# Autodesk Inventor assembly: Motor assembly
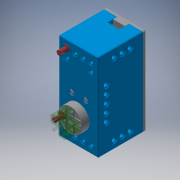
[picture p0: Inventor's stored thumbnail of the model, 180x180]
Saved by Autodesk Inventor 2019 (Build 230136000, 136)
## iProperties
Created: 2018-11-22
Part Number: Motor assembly
Document SubType Name: Assembly
Designer: Varga Daniel
Author: Varga Daniel
## Documents named in this file (11)
- C:\!_Dani\!_cloud\OneDrive\!_munka\Revolution\RevvyDemoKit\Structural parts\Demo parts\Motor\Motor assembly.iam
- C:\!_Dani\!_cloud\OneDrive\!_munka\Revolution\RevvyDemoKit\Structural parts\Demo parts\Motor\FIT0450 motor\FIT0450.iam
- C:\!_Dani\!_cloud\OneDrive\!_munka\Revolution\RevvyDemoKit\Structural parts\Connetor Pins\cp1x1.ipt
- C:\!_Dani\!_cloud\OneDrive\!_munka\Revolution\RevvyDemoKit\Structural parts\Axle Connectors\Axle connector 3x3 cross.ipt
- C:\!_Dani\!_cloud\OneDrive\!_munka\Revolution\RevvyDemoKit\Structural parts\Demo parts\Motor\Motor rotor.ipt
- C:\!_Dani\!_cloud\OneDrive\!_munka\Revolution\RevvyDemoKit\Structural parts\Axles\Axle 2.ipt
- C:\!_Dani\!_cloud\OneDrive\!_dokumentumok\Inventor\Content Center Files\R2019\en-US\ISO 1207(2)\ISO 1207 - M3 x 6.ipt
- C:\!_Dani\!_cloud\OneDrive\!_munka\Revolution\RevvyDemoKit\Structural parts\Demo parts\Motor\Motor cover lower.ipt
- C:\!_Dani\!_cloud\OneDrive\!_dokumentumok\Inventor\Content Center Files\R2019\en-US\ISO 4032(2)\ISO 4032 - M2,5 - ISO.ipt
- C:\!_Dani\!_cloud\OneDrive\!_dokumentumok\Inventor\Content Center Files\R2019\en-US\DIN 7985 (H)\DIN 7985 (H) - M2,5x30-H.ipt
- C:\!_Dani\!_cloud\OneDrive\!_munka\Revolution\RevvyDemoKit\Structural parts\Demo parts\Motor\Motor cover upper.ipt
## Components (15 placed, 10 different names)
1. FIT0450:1 [sub-assembly] — Mate:7, Angle:1, Mate:8, Mate:15, Mate:16, Mate:17, Mate:18, Mate:19, Angle:2
2. cp1x1:1 — Mate:2, Mate:3, Mate:4, Mate:5
3. Axle connector 3x3 cross:1 — Mate:2, Mate:3, Mate:6, Mate:10, Mate:11
4. Motor rotor:1 — Mate:4, Mate:5, Mate:6, Mate:7, Angle:1, Mate:8, Mate:12, Mate:13, Mate:14, Mate:15
5. Axle 2:1 — Mate:10, Mate:11, Mate:14
6. ISO 1207 M3 x 6:1 — Mate:12, Mate:13
7. ISO 4032 M2,5:1 — Mate:16, Mate:17, Flush:2, Flush:3, Angle:2, Angle:3, Angle:4, Flush:4, Mate:20
8. ISO 4032 M2,5:2 — Flush:2, Mate:18, Angle:3, Mate:21, Flush:5
9. ISO 4032 M2,5:3 — Flush:3, Mate:19, Angle:4, Mate:22, Flush:6, Flush:7
10. DIN 7985 (H) M2,5x30-H:1 — Flush:4, Mate:20
11. DIN 7985 (H) M2,5x30-H:2 — Mate:21, Flush:5, Mate:24
12. DIN 7985 (H) M2,5x30-H:3 — Mate:22, Flush:6, Mate:23
13. cp1x1:2 — Mate:26, Mate:27, Mate:28
14. Motor cover lower:1 — Flush:7, Mate:23, Mate:24, Mate:25, Mate:26, Mate:27, Mate:28
15. Motor cover upper:1 — Mate:25
## Relationships (36: Mate 26, Flush 6, Angle 4)
- Mate:2: cp1x1:1 ↔ Axle connector 3x3 cross:1
- Mate:3: cp1x1:1 ↔ Axle connector 3x3 cross:1
- Mate:4: cp1x1:1 ↔ Motor rotor:1
- Mate:5: cp1x1:1 ↔ Motor rotor:1
- Mate:6: Axle connector 3x3 cross:1 ↔ Motor rotor:1
- Mate:7: FIT0450:1 ↔ Motor rotor:1
- Angle:1 (0 deg): FIT0450:1 ↔ Motor rotor:1
- Mate:8: FIT0450:1 ↔ Motor rotor:1
- Mate:10: Axle connector 3x3 cross:1 ↔ Axle 2:1
- Mate:11: Axle connector 3x3 cross:1 ↔ Axle 2:1
- Mate:12: Motor rotor:1 ↔ ISO 1207 M3 x 6:1
- Mate:13: Motor rotor:1 ↔ ISO 1207 M3 x 6:1
- Mate:14: Motor rotor:1 ↔ Axle 2:1
- Mate:15: FIT0450:1 ↔ Motor rotor:1
- Mate:16: FIT0450:1 ↔ ISO 4032 M2,5:1
- Mate:17 (3.5 mm): FIT0450:1 ↔ ISO 4032 M2,5:1
- Flush:2: ISO 4032 M2,5:1 ↔ ISO 4032 M2,5:2
- Mate:18: FIT0450:1 ↔ ISO 4032 M2,5:2
- Flush:3: ISO 4032 M2,5:1 ↔ ISO 4032 M2,5:3
- Mate:19: FIT0450:1 ↔ ISO 4032 M2,5:3
- Angle:2 (0 deg): FIT0450:1 ↔ ISO 4032 M2,5:1
- Angle:3 (0 deg): ISO 4032 M2,5:1 ↔ ISO 4032 M2,5:2
- Angle:4 (0 deg): ISO 4032 M2,5:1 ↔ ISO 4032 M2,5:3
- Flush:4: ISO 4032 M2,5:1 ↔ DIN 7985 (H) M2,5x30-H:1
- Mate:20: ISO 4032 M2,5:1 ↔ DIN 7985 (H) M2,5x30-H:1
- Mate:21: ISO 4032 M2,5:2 ↔ DIN 7985 (H) M2,5x30-H:2
- Flush:5: ISO 4032 M2,5:2 ↔ DIN 7985 (H) M2,5x30-H:2
- Mate:22: ISO 4032 M2,5:3 ↔ DIN 7985 (H) M2,5x30-H:3
- Flush:6: ISO 4032 M2,5:3 ↔ DIN 7985 (H) M2,5x30-H:3
- Flush:7: ISO 4032 M2,5:3 ↔ Motor cover lower:1
- Mate:23: DIN 7985 (H) M2,5x30-H:3 ↔ Motor cover lower:1
- Mate:24: DIN 7985 (H) M2,5x30-H:2 ↔ Motor cover lower:1
- Mate:25 (-60 mm): Motor cover lower:1 ↔ Motor cover upper:1
- Mate:26 (-10 mm): cp1x1:2 ↔ Motor cover lower:1
- Mate:27 (-10 mm): cp1x1:2 ↔ Motor cover lower:1
- Mate:28: cp1x1:2 ↔ Motor cover lower:1
